# Autodesk Inventor assembly: M178-PHTM-3000-03
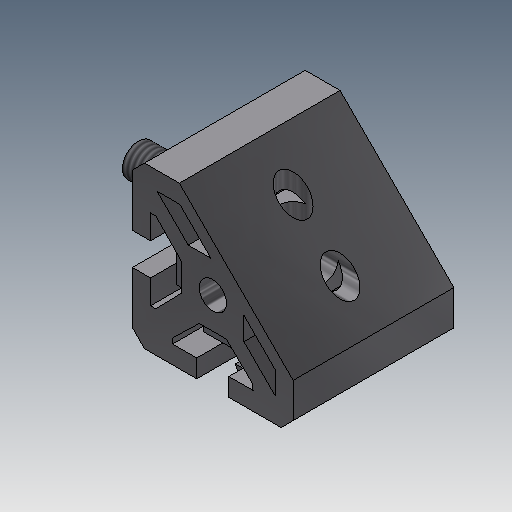
[picture p0: Inventor's stored thumbnail of the model, 512x512]
Saved by Autodesk Inventor 2018.3 (Build 223284000, 284)
## iProperties
Created: 2004-11-23
Part Number: M178-PHTM-3000-03
Document SubType Name: Assembly
Designer: Autodesk, Inc.
Manufacturer: Standard
Standards Organization: Custom
Description: PHANTOM, CORNER BRACKET 2
Mass: 127.896 g
Surface Area: 191.467 cm^2
Volume: 35.6746 cm^3
Density: 3.58509 g/cm^3
CAGE: 1LJX3
Dept. ID: Product Design
Description #2: ---
Finish #1: ---
Finish #2: ---
Material ID: ---
Project Number: ---
Author: Autodesk, Inc.
## Documents named in this file (9)
- C:\AVAInvAPI\Workspace\Test Station\Components\21-135 Corner Phantom 2.iam
- C:\AVAInvAPI\Workspace\Test Station\Components\21-135.ipt
- C:\AVAInvAPI\Workspace\Test Station\Components\20-028.iam
- C:\AVAInvAPI\Workspace\Test Station\Components\20-058.ipt
- C:\AVAInvAPI\Workspace\Test Station\Components\20-028Z1.ipt
- C:\AVAInvAPI\Workspace\Test Station\Components\24-125-8.ipt
- C:\Users\kelleyb.ADS\Desktop\Samples MIGRATED 2009 224 RTM_1\Standard Parts\Test Station Content\Corners, Gussets, and Mounting Plates\21-XXX Corner Elements.ipt
- C:\Users\kelleyb.ADS\Desktop\Samples MIGRATED 2009 224 RTM_1\Standard Parts\Test Station Content\Fastners\20-XXX TSlot Nuts.ipt
- C:\Users\kelleyb.ADS\Desktop\Samples MIGRATED 2009 224 RTM_1\Standard Parts\Test Station Content\Fastners\2X-YYY-ZZ IPS Screws.ipt
## Components (5 placed, 5 different names)
1. 21-135:1 — Mate:3, Mate:4, Angle:2, Mate:7, Angle:4, Mate:8, Mate:9, Angle:5
2. 20-028:2 [sub-assembly] — Mate:3, Mate:4, Angle:2, Mate:6
3. 20-058:2 — Mate:6, Mate:7, Angle:4
4. 20-028Z1:1 — Insert:1, Mate:9, Angle:5
5. 24-125-8:1 — Insert:1, Mate:8
## Relationships (10: Mate 6, Angle 3, Insert 1)
- Mate:3: 21-135:1 ↔ 20-028:2
- Mate:4: 21-135:1 ↔ 20-028:2
- Angle:2 (0 deg): 21-135:1 ↔ 20-028:2
- Mate:6: 20-028:2 ↔ 20-058:2
- Mate:7 (4.5 mm): 21-135:1 ↔ 20-058:2
- Angle:4 (0 deg): 21-135:1 ↔ 20-058:2
- Insert:1: 20-028Z1:1 ↔ 24-125-8:1
- Mate:8: 21-135:1 ↔ 24-125-8:1
- Mate:9: 21-135:1 ↔ 20-028Z1:1
- Angle:5 (0 deg): 21-135:1 ↔ 20-028Z1:1
